# Autodesk Inventor assembly: GATITOLOCOV2
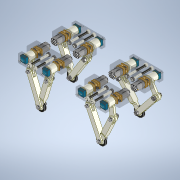
[picture p0: Inventor's stored thumbnail of the model, 180x180]
Saved by Autodesk Inventor 2022 (Build 260153000, 153)
## iProperties
Created: 2021-11-23
Part Number: GATITOLOCOV2
Document SubType Name: Assembly
Designer: JK
Author: JK
## Documents named in this file (2)
- C:\Users\JK\Documents\Inventor\N20 Leg Actuator\CADfiles\GATITOLOCOV2.iam
- C:\Users\JK\Documents\Inventor\N20 Leg Actuator\CADfiles\Leg Assembly (small bearing).iam
## Components (4 placed, 1 different names)
1. Leg Assembly (small bearing):1 [sub-assembly] — Coincidencia:2, Nivelación:3, Nivelación:4, Nivelación:5, Nivelación:6
2. Leg Assembly (small bearing):2 [sub-assembly] — Nivelación:5, Nivelación:6, Nivelación:7
3. Leg Assembly (small bearing):3 [sub-assembly] — Coincidencia:1, Nivelación:1, Nivelación:2, Coincidencia:2, Nivelación:3, Nivelación:4
4. Leg Assembly (small bearing):4 [sub-assembly] — Coincidencia:1, Nivelación:1, Nivelación:2, Nivelación:7
## Relationships (9: Flush 7, Mate 2)
- Coincidencia:1 [Mate] (40 mm): Leg Assembly (small bearing):3 ↔ Leg Assembly (small bearing):4
- Nivelación:1 [Flush]: Leg Assembly (small bearing):3 ↔ Leg Assembly (small bearing):4
- Nivelación:2 [Flush]: Leg Assembly (small bearing):3 ↔ Leg Assembly (small bearing):4
- Coincidencia:2 [Mate] (30 mm): Leg Assembly (small bearing):1 ↔ Leg Assembly (small bearing):3
- Nivelación:3 [Flush]: Leg Assembly (small bearing):1 ↔ Leg Assembly (small bearing):3
- Nivelación:4 [Flush]: Leg Assembly (small bearing):1 ↔ Leg Assembly (small bearing):3
- Nivelación:5 [Flush]: Leg Assembly (small bearing):1 ↔ Leg Assembly (small bearing):2
- Nivelación:6 [Flush]: Leg Assembly (small bearing):1 ↔ Leg Assembly (small bearing):2
- Nivelación:7 [Flush]: Leg Assembly (small bearing):2 ↔ Leg Assembly (small bearing):4
